# Autodesk Inventor assembly: МД.001.600 - Звено 2
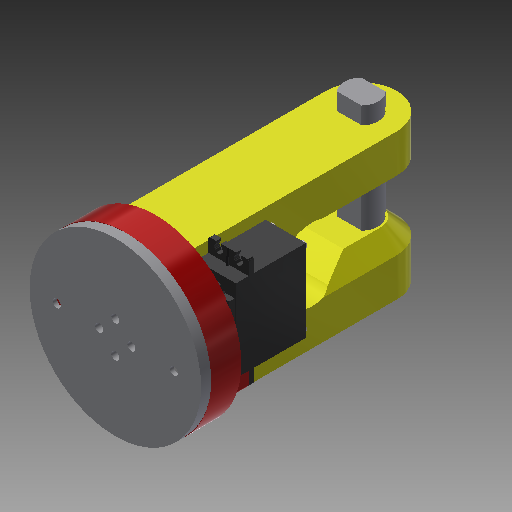
[picture p0: Inventor's stored thumbnail of the model, 512x512]
Saved by Autodesk Inventor 2019 (Build 230136000, 136)
## iProperties
Created: 2019-12-29
Part Number: МД.001.600 - Звено 2
Material: Типовые
Document SubType Name: Assembly
Designer: Петров Иван
Author: Петров Иван
## Documents named in this file (4)
- E:\IVAN\Ivan_desktop\GitHub\Arm_manip\hardware\new\МД.001.600 - Звено 2.iam
- E:\IVAN\Ivan_desktop\GitHub\Arm_manip\hardware\new\МД.001.601 - Ось звена 2.ipt
- E:\IVAN\Ivan_desktop\GitHub\Arm_manip\hardware\new\МД.001.602 - Начало звена 2.ipt
- E:\IVAN\Ivan_desktop\GitHub\Arm_manip\hardware\new\МД.001.700 - Поворотный механизм.iam
## Components (3 placed, 3 different names)
1. МД.001.601 - Ось звена 2:1 — Совмещение:1, Совмещение:2, Заподлицо:1
2. МД.001.602 - Начало звена 2:1 — Совмещение:1, Совмещение:2, Заподлицо:1, Совмещение:3, Совмещение:4, Совмещение:5
3. МД.001.700 - Поворотный механизм:1 [sub-assembly] — Совмещение:3, Совмещение:4, Совмещение:5
## Relationships (6: Mate 5, Flush 1)
- Совмещение:1 [Mate]: МД.001.601 - Ось звена 2:1 ↔ МД.001.602 - Начало звена 2:1
- Совмещение:2 [Mate]: МД.001.601 - Ось звена 2:1 ↔ МД.001.602 - Начало звена 2:1
- Заподлицо:1 [Flush] (8.4 mm): МД.001.601 - Ось звена 2:1 ↔ МД.001.602 - Начало звена 2:1
- Совмещение:3 [Mate]: МД.001.602 - Начало звена 2:1 ↔ МД.001.700 - Поворотный механизм:1
- Совмещение:4 [Mate]: МД.001.602 - Начало звена 2:1 ↔ МД.001.700 - Поворотный механизм:1
- Совмещение:5 [Mate]: МД.001.602 - Начало звена 2:1 ↔ МД.001.700 - Поворотный механизм:1
